# Autodesk Inventor assembly: ABD_Version_0.1_leftleg
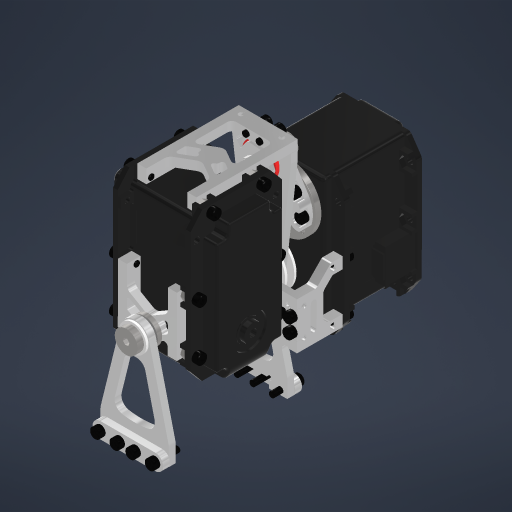
[picture p0: Inventor's stored thumbnail of the model, 512x512]
Saved by Autodesk Inventor 2024.3 (Build 283343000, 343)
## iProperties
Created: 2024-01-23
Part Number: ABD_Version_0.1_leftleg
Document SubType Name: Assembly
Designer: ASUS
Mass: 357.136 g
Surface Area: 604.848 cm^2
Volume: 181.423 cm^3
Density: 1.96853 g/cm^3
Author: ASUS
## Documents named in this file (6)
- C:\Users\ASUS\Desktop\Anti_Backlash_Structure_OP\v2_Frame\ABD_V2_Left_OP.iam
- C:\Users\ASUS\Desktop\ABD_2024_Eindhoven\MISUMI\Crank_Slider_Fixer.iam
- C:\Users\ASUS\Desktop\Anti_Backlash_Structure_OP\v2_Frame\Roll_Fixation_Set.iam
- C:\Users\ASUS\Desktop\Anti_Backlash_Structure_OP\v2_Frame\ABD_MX_64_Roll_Fixation_Set.iam
- C:\Users\ASUS\Desktop\Anti_Backlash_Structure_OP\v2_Frame\ABD_MX_64_Slider_Fixation_Set_Right2Horn.iam
- C:\Users\ASUS\Desktop\Anti_Backlash_Structure_OP\v2_Frame\ABD_Slider_Set_v2.iam
## Components (5 placed, 5 different names)
1. ABD_Slider_Set_v2:1 [sub-assembly]
2. Roll_Fixation_Set:1 [sub-assembly] — 삽입:4, 삽입:5
3. Crank_Slider_Fixer:1 [sub-assembly]
4. ABD_MX_64_Roll_Fixation_Set:1 [sub-assembly] — 메이트:2, 메이트:3, 삽입:5
5. ABD_MX_64_Slider_Fixation_Set_Right2Horn:1 [sub-assembly] — 삽입:4, 메이트:2, 메이트:3
## Relationships (6: Insert 4, Mate 2)
- [Insert]: ABD_Slider_Set_v2:1 ↔ Roll_Fixation_Set:1
- [Insert]: ABD_Slider_Set_v2:1 ↔ Crank_Slider_Fixer:1
- 삽입:4 [Insert]: Roll_Fixation_Set:1 ↔ ABD_MX_64_Slider_Fixation_Set_Right2Horn:1
- 메이트:2 [Mate] (0.05 mm): ABD_MX_64_Roll_Fixation_Set:1 ↔ ABD_MX_64_Slider_Fixation_Set_Right2Horn:1
- 메이트:3 [Mate]: ABD_MX_64_Roll_Fixation_Set:1 ↔ ABD_MX_64_Slider_Fixation_Set_Right2Horn:1
- 삽입:5 [Insert]: Roll_Fixation_Set:1 ↔ ABD_MX_64_Roll_Fixation_Set:1
